# Autodesk Inventor assembly: PossibleClaw1
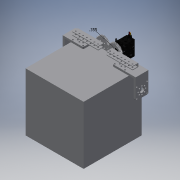
[picture p0: Inventor's stored thumbnail of the model, 180x180]
Saved by Autodesk Inventor 2017 (Build 210142000, 142)
## iProperties
Created: 2017-09-20
Part Number: PossibleClaw1
Document SubType Name: Assembly
Designer: User
Author: User
## Documents named in this file (6)
- C:\Robotics\CAD\2017-18_CAD\PossibleClaw1.iam
- C:\Robotics\CAD\2017-18_CAD\Glyph6x6x6.ipt
- C:\Robotics\CAD\COTSParts\Tetrix\Tetrix 180 Servo.ipt
- C:\Robotics\CAD\COTSParts\Actobotics\585 parts\585494.ipt
- C:\Robotics\CAD\COTSParts\Actobotics\585 parts\585382.ipt
- C:\Robotics\CAD\COTSParts\Tetrix\Tetrix Gear 40T.ipt
## Components (8 placed, 5 different names)
1. Glyph6x6x6:1 — Mate:1, Flush:4, Mate:2
2. Tetrix 180 Servo:1 — Insert:8
3. 585494:1 — Flush:3, Insert:7, Flush:4, Mate:2
4. 585494:2 — Flush:3, Insert:1, Insert:2, Mate:1
5. 585382:2 — Insert:5, Insert:7
6. 585382:3 — Insert:1, Insert:2, Insert:6
7. Tetrix Gear 40T:1 — Insert:6, Tangent:1
8. Tetrix Gear 40T:2 — Insert:5, Tangent:1, Insert:8
## Relationships (11: Insert 6, Flush 2, Mate 2, Tangent 1)
- Flush:3: 585494:1 ↔ 585494:2
- Insert:1: 585494:2 ↔ 585382:3
- Insert:2: 585494:2 ↔ 585382:3
- Insert:5: 585382:2 ↔ Tetrix Gear 40T:2
- Insert:6: 585382:3 ↔ Tetrix Gear 40T:1
- Tangent:1: Tetrix Gear 40T:1 ↔ Tetrix Gear 40T:2
- Insert:7: 585494:1 ↔ 585382:2
- Insert:8: Tetrix 180 Servo:1 ↔ Tetrix Gear 40T:2
- Mate:1: Glyph6x6x6:1 ↔ 585494:2
- Flush:4: Glyph6x6x6:1 ↔ 585494:1
- Mate:2 (12.7 mm): Glyph6x6x6:1 ↔ 585494:1
